# Autodesk Inventor assembly: Orienter_Assembly
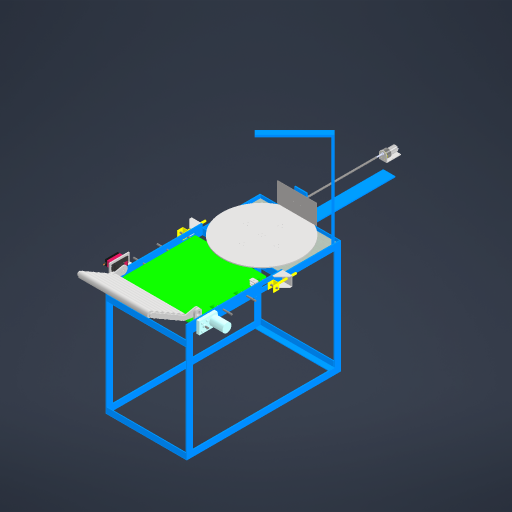
[picture p0: Inventor's stored thumbnail of the model, 512x512]
Saved by Autodesk Inventor 2023 (Build 270158000, 158)
## iProperties
Created: 2023-11-04
Part Number: Orienter_Assembly
Document SubType Name: Assembly
Designer: Abhinav
Author: Abhinav
## Documents named in this file (15)
- C:\Users\Abhinav\Desktop\GRID\ARM 3\Orienter\Orienter_Assembly.iam
- C:\Users\Abhinav\Desktop\GRID\ARM 3\Orienter\Conveyor.ipt
- C:\Users\Abhinav\Desktop\GRID\ARM 3\Orienter\Structure.ipt
- C:\Users\Abhinav\Desktop\3D Library\Rectangular-Motor.ipt
- C:\Users\Abhinav\Desktop\3D Library\60 kg cm Servo.ipt
- C:\Users\Abhinav\Desktop\GRID\ARM 3\Orienter\Base.ipt
- C:\Users\Abhinav\Desktop\GRID\ARM 3\Orienter\Servo_fix.ipt
- C:\Users\Abhinav\Desktop\GRID\ARM 3\Orienter\Bear_fix.ipt
- C:\Users\Abhinav\Desktop\GRID\ARM 3\Orienter\Orienter.ipt
- C:\Users\Abhinav\Desktop\GRID\ARM 3\Orienter\Servo_horn_big.ipt
- C:\Users\Abhinav\Desktop\GRID\ARM 3\Orienter\Tensioner.ipt
- C:\Users\Abhinav\Desktop\GRID\ARM 3\Orienter\Tensioner_fix.ipt
- C:\Users\Abhinav\Desktop\GRID\ARM 3\Orienter\Align_Roller.ipt
- C:\Users\Abhinav\Desktop\GRID\ARM 3\Orienter\Aligner.ipt
- C:\Users\Abhinav\Desktop\GRID\ARM 3\Orienter\Push.iam
## Components (18 placed, 14 different names)
1. Conveyor:1 — Mate:3, Mate:24, Flush:3, Mate:32, Mate:33, Mate:35, Mate:41
2. Structure:1 — Mate:3, Mate:4, Mate:5, Mate:6, Mate:17, Mate:18, Mate:19, Mate:23, Mate:37, Mate:38, Mate:39, Mate:41, Mate:42, Mate:43, Flush:6, Flush:7, Mate:46, Flush:8, Flush:9, Mate:48, Mate:49, Mate:50, Mate:55, Angle:1
3. Rectangular-Motor:1 — Mate:4, Mate:5, Mate:6, Mate:25, Mate:32
4. Base:1 — Mate:40, Mate:42
5. Servo_fix:1 — Mate:17, Mate:18, Mate:19, Mate:20, Mate:21, Mate:22, Flush:5
6. 60 kg cm Servo:2 — Mate:20, Mate:21, Mate:22, Flush:2, Mate:26, Mate:31
7. Bear_fix:1 — Mate:23, Mate:24, Mate:25
8. Orienter:1 — Mate:26, Mate:27, Flush:3
9. Servo_horn_big:1 — Mate:31, Flush:5, Mate:27
10. Tensioner:1 — Mate:33, Mate:47
11. Tensioner:2 — Mate:35, Mate:44
12. Rectangular-Motor:2 — Mate:37, Mate:38, Mate:39, Mate:40
13. Tensioner_fix:1 — Mate:43, Flush:6, Flush:7, Mate:44
14. Tensioner_fix:2 — Mate:46, Flush:8, Flush:9, Mate:47
15. Align_Roller:1 — Mate:53, Mate:54
16. Aligner:1 — Mate:48, Mate:49, Mate:50, Mate:51, Mate:52, Mate:53, Mate:54
17. Align_Roller:2 — Mate:51, Mate:52
18. Push:1 [sub-assembly] — Mate:55, Angle:1
## Relationships (45: Mate 37, Flush 7, Angle 1)
- Mate:3 (25 mm): Conveyor:1 ↔ Structure:1
- Mate:4: Structure:1 ↔ Rectangular-Motor:1
- Mate:5: Structure:1 ↔ Rectangular-Motor:1
- Mate:6: Structure:1 ↔ Rectangular-Motor:1
- Mate:17 (15 mm): Structure:1 ↔ Servo_fix:1
- Mate:18: Structure:1 ↔ Servo_fix:1
- Mate:19: Structure:1 ↔ Servo_fix:1
- Mate:20: Servo_fix:1 ↔ 60 kg cm Servo:2
- Mate:21: Servo_fix:1 ↔ 60 kg cm Servo:2
- Mate:22: Servo_fix:1 ↔ 60 kg cm Servo:2
- Flush:2: 60 kg cm Servo:2
- Mate:23: Structure:1 ↔ Bear_fix:1
- Mate:24: Conveyor:1 ↔ Bear_fix:1
- Mate:25: Rectangular-Motor:1 ↔ Bear_fix:1
- Mate:26: 60 kg cm Servo:2 ↔ Orienter:1
- Mate:27 (5 mm): Orienter:1 ↔ Servo_horn_big:1
- Flush:3: Conveyor:1 ↔ Orienter:1
- Mate:31: 60 kg cm Servo:2 ↔ Servo_horn_big:1
- Flush:5 (-30 mm): Servo_fix:1 ↔ Servo_horn_big:1
- Mate:32: Conveyor:1 ↔ Rectangular-Motor:1
- Mate:33: Conveyor:1 ↔ Tensioner:1
- Mate:35: Conveyor:1 ↔ Tensioner:2
- Mate:37: Structure:1 ↔ Rectangular-Motor:2
- Mate:38: Structure:1 ↔ Rectangular-Motor:2
- Mate:39: Structure:1 ↔ Rectangular-Motor:2
- Mate:40: Base:1 ↔ Rectangular-Motor:2
- Mate:41: Conveyor:1 ↔ Structure:1
- Mate:42 (30 mm): Structure:1 ↔ Base:1
- Mate:43: Structure:1 ↔ Tensioner_fix:1
- Flush:6: Structure:1 ↔ Tensioner_fix:1
- Flush:7: Structure:1 ↔ Tensioner_fix:1
- Mate:44: Tensioner:2 ↔ Tensioner_fix:1
- Mate:46: Structure:1 ↔ Tensioner_fix:2
- Flush:8: Structure:1 ↔ Tensioner_fix:2
- Flush:9: Structure:1 ↔ Tensioner_fix:2
- Mate:47: Tensioner:1 ↔ Tensioner_fix:2
- Mate:48: Structure:1 ↔ Aligner:1
- Mate:49: Structure:1 ↔ Aligner:1
- Mate:50: Structure:1 ↔ Aligner:1
- Mate:51 (5 mm): Aligner:1 ↔ Align_Roller:2
- Mate:52: Aligner:1 ↔ Align_Roller:2
- Mate:53 (5 mm): Align_Roller:1 ↔ Aligner:1
- Mate:54: Align_Roller:1 ↔ Aligner:1
- Mate:55: Structure:1 ↔ Push:1
- Angle:1 (0 deg): Structure:1 ↔ Push:1
